# Autodesk Inventor assembly: Assembly1
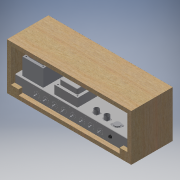
[picture p0: Inventor's stored thumbnail of the model, 180x180]
Saved by Autodesk Inventor 2016 (Build 200138000, 138)
## iProperties
Created: 2015-10-14
Part Number: Assembly1
Document SubType Name: Assembly
Designer: jeremyhale
Author: jeremyhale
## Documents named in this file (22)
- \\psf\Home\Documents\Poorhouse\git\p0001\Assembly1.iam
- \\psf\Home\Documents\Poorhouse\git\p0001\chassis.ipt
- \\psf\Home\Documents\Poorhouse\git\p0001\tube socket 8 pin.ipt
- \\psf\Home\Documents\Poorhouse\git\p0001\tube socket 9 pin.ipt
- \\psf\Home\Documents\Poorhouse\git\p0001\xmfr power.ipt
- \\psf\Home\Documents\Poorhouse\git\p0001\xmfr output.ipt
- \\psf\Home\Documents\Inventor\Content Center Files\R2016\en-US\AS 1427(08)\AS 1427 - M3 x 5(6) I.ipt
- \\psf\Home\Documents\Inventor\Content Center Files\R2016\en-US\AS 1474(1)\AS 1474 - M2.5(1).ipt
- \\psf\Home\Documents\Inventor\Content Center Files\R2016\en-US\AS 1474(1)\AS 1474 - M3.5(1).ipt
- \\psf\Home\Documents\Inventor\Content Center Files\R2016\en-US\AS 1474(1)\AS 1474 - M3(1).ipt
- \\psf\Home\Documents\Poorhouse\git\p0001\cabinet.ipt
- \\psf\Home\Documents\Poorhouse\git\p0001\iec320_703W-00_04.ipt
- \\psf\Home\Documents\Inventor\Content Center Files\R2016\en-US\AS 1427(07)\AS 1427 - M3 x 10(6) II.ipt
- \\psf\Home\Documents\Poorhouse\git\p0001\Toggle Large A.ipt
- \\psf\Home\Documents\Poorhouse\git\p0001\AUDIO JACK 2.ipt
- \\psf\Home\Documents\Poorhouse\git\p0001\12ax7_complete.ipt
- \\psf\Home\Documents\Poorhouse\git\p0001\Noval socket.ipt
- \\psf\Home\Documents\Poorhouse\git\p0001\octal assembly.ipt
- \\psf\Home\Documents\Poorhouse\git\p0001\el34 assembly_r1.ipt
- \\psf\Home\Documents\Poorhouse\git\p0001\rotary control.iam
- \\psf\Home\Documents\Poorhouse\git\p0001\Bussman fuse holder HKP - 0,25'' X 1,25''.ipt
- \\psf\Home\Documents\Poorhouse\git\p0001\cage nut m6.ipt
## Components (94 placed, 25 different names)
1. chassis:1 — Rotational:1, Rotational:2, Rotational:3, Rotational:4, Rotational:5, Rotational:6, Rotational:7, Rotational:8, Rotational:9, Rotational:10, Mate:4, Insert:20, Insert:21, Insert:22, Insert:23, Insert:24, Insert:25, Insert:26, Insert:27, Insert:28, Insert:29, Insert:30, Insert:31, Insert:32, Insert:33, Insert:34, Insert:35, Insert:36, Insert:37, Flush:1, Mate:5, Flush:2, Rotational:11, Rotational:12, Mate:11, Mate:13, Rigid:15, Rigid:18, Rigid:19, Rigid:20, Rotational:15, Rotational:16, Rotational:17, Rotational:18, Rotational:19, Rotational:20, Rotational:26, Rotational:27, Rigid:22, Rigid:23, Rigid:24, Rigid:25, Rigid:26
2. big preamp tube sockets — Rotational:3, Rotational:4, Insert:13, Insert:14
3. xmfr power:1 — Rotational:7, Rotational:8
4. xmfr output:1 — Rotational:9, Rotational:10
5. cabinet:1 — Flush:1, Mate:5, Flush:2
6. PowerSwitch — Rigid:23
7. Bussman fuse holder HKP - 0,25'' X 1,25'':1 — Rigid:22
8. Input Jack — Rotational:26
9. AS 1427 Z - Metric M3 x 5:1 — Insert:1, Mate:3
10. AS 1427 Z - Metric M3 x 5:2 — Insert:2
11. AS 1427 Z - Metric M3 x 5:3 — Insert:3
12. AS 1427 Z - Metric M3 x 5:4 — Insert:4
13. AS 1427 Z - Metric M3 x 5:5 — Insert:5
14. AS 1427 Z - Metric M3 x 5:6 — Insert:6
15. AS 1427 Z - Metric M3 x 5:7 — Insert:7
16. AS 1427 Z - Metric M3 x 5:8 — Insert:8
17. AS 1427 Z - Metric M3 x 5:9 — Insert:9
18. AS 1427 Z - Metric M3 x 5:10 — Insert:10
19. AS 1427 Z - Metric M3 x 5:11 — Insert:11
20. AS 1427 Z - Metric M3 x 5:12 — Insert:12
21. AS 1427 Z - Metric M3 x 5:13 — Insert:13
22. AS 1427 Z - Metric M3 x 5:14 — Insert:14
23. AS 1427 Z - Metric M3 x 5:15 — Insert:15
24. AS 1427 Z - Metric M3 x 5:16 — Insert:16
25. AS 1427 Z - Metric M3 x 5:17 — Insert:17
26. AS 1427 Z - Metric M3 x 5:18 — Insert:18
27. AS 1474 - Metric M2.5:1 — Mate:3, Mate:4
28. AS 1474 - Metric M3.5:1 — Insert:20
29. AS 1474 - Metric M3.5:2 — Insert:21
30. AS 1474 - Metric M3.5:3 — Insert:22
31. AS 1474 - Metric M3.5:4 — Insert:23
32. AS 1474 - Metric M3.5:5 — Insert:24
33. AS 1474 - Metric M3.5:6 — Insert:25
34. AS 1474 - Metric M3.5:7 — Insert:26
35. AS 1474 - Metric M3.5:8 — Insert:27
36. AS 1474 - Metric M3.5:9 — Insert:28
37. AS 1474 - Metric M3.5:10 — Insert:29
38. AS 1474 - Metric M3.5:11 — Insert:30
39. AS 1474 - Metric M3.5:12 — Insert:31
40. AS 1474 - Metric M3.5:13 — Insert:32
41. AS 1474 - Metric M3.5:14 — Insert:33
42. AS 1474 - Metric M3:1 — Insert:34
43. AS 1474 - Metric M3:2 — Insert:35
44. AS 1474 - Metric M3:3 — Insert:36
45. AS 1474 - Metric M3:4 — Insert:37
46. iec320_703W-00_04:1 — Rotational:11, Rotational:12, Mate:6, Mate:7
47. AS 1427 Z - Metric M3 x 10:2 — Mate:6, Mate:10
48. AS 1427 Z - Metric M3 x 10:1 — Mate:7, Mate:12
49. AS 1474 - Metric M3:5 — Mate:10, Mate:11
50. AS 1474 - Metric M3:6 — Mate:12, Mate:13
51. 12ax7_complete:1 — Rotational:13
52. 12ax7_complete:2 — Rotational:14
53. Noval socket:1 — Rigid:18, Rotational:13
54. Noval socket:2 — Rigid:19, Rotational:14
55. octal assembly:1 — Rigid:20
56. octal assembly:2 — Rotational:15, Rotational:21
57. octal assembly:3 — Rotational:16, Rotational:22
58. octal assembly:4 — Rotational:18, Rotational:23
59. octal assembly:5 — Rotational:17, Rigid:21
60. octal assembly:6 — Rotational:19, Rotational:24
61. octal assembly:7 — Rotational:20, Rotational:25
62. el34 assembly_r1:1 — Rotational:21
63. el34 assembly_r1:2 — Rotational:22
64. el34 assembly_r1:3 — Rigid:21
65. el34 assembly_r1:4 — Rotational:23
66. el34 assembly_r1:5 — Rotational:24
67. el34 assembly_r1:6 — Rotational:25
68. tube socket 8 pin:1 — Rotational:1, Rotational:2, Insert:1, Insert:2
69. tube socket 8 pin:2 — Insert:3, Insert:4
70. tube socket 8 pin:3 — Insert:5, Insert:6
71. tube socket 8 pin:4 — Insert:7, Insert:8
72. tube socket 8 pin:5 — Insert:15, Insert:16
73. tube socket 8 pin:6 — Insert:17, Insert:18
74. tube socket 9 pin:1 — Rotational:5, Rotational:6, Insert:9, Insert:10
75. tube socket 9 pin:2 — Insert:11, Insert:12
76. rotary control:1 [sub-assembly] — Rotational:27
77. rotary control:2 [sub-assembly]
78. rotary control:3 [sub-assembly]
79. rotary control:4 [sub-assembly]
80. rotary control:5 [sub-assembly]
81. rotary control:6 [sub-assembly]
82. rotary control:7 [sub-assembly]
83. rotary control:8 [sub-assembly]
84. Speaker — Rigid:15
85. AUDIO JACK 2:3
86. AUDIO JACK 2:4
87. cage nut cage — Rigid:24
88. cage nut m6:2
89. cage nut m6:3
90. cage nut m6:4
91. cage nut m6:5 — Rigid:25
92. cage nut m6:6
93. cage nut m6:7 — Rigid:26
94. cage nut m6:8
## Component patterns: Big Tube Sockets (6 elements), small preamp tube sockets (2 elements), Rotary Controls (8 elements), Speaker Jacks (3 elements), Cage Nuts Top (4 elements), Cage Nuts Side Right (2 elements), Cage Nuts Side Left (2 elements)
## Relationships (84: Insert 36, RevoluteJoint 27, WeldJoint 10, Mate 9, Flush 2)
- Rotational:1 [RevoluteJoint]: chassis:1 ↔ tube socket 8 pin:1
- Rotational:2 [RevoluteJoint]: chassis:1 ↔ tube socket 8 pin:1
- Rotational:3 [RevoluteJoint]: chassis:1 ↔ big preamp tube sockets
- Rotational:4 [RevoluteJoint]: chassis:1 ↔ big preamp tube sockets
- Rotational:5 [RevoluteJoint]: chassis:1 ↔ tube socket 9 pin:1
- Rotational:6 [RevoluteJoint]: chassis:1 ↔ tube socket 9 pin:1
- Rotational:7 [RevoluteJoint]: chassis:1 ↔ xmfr power:1
- Rotational:8 [RevoluteJoint]: chassis:1 ↔ xmfr power:1
- Rotational:9 [RevoluteJoint]: chassis:1 ↔ xmfr output:1
- Rotational:10 [RevoluteJoint]: chassis:1 ↔ xmfr output:1
- Insert:1: AS 1427 Z - Metric M3 x 5:1 ↔ tube socket 8 pin:1
- Insert:2: AS 1427 Z - Metric M3 x 5:2 ↔ tube socket 8 pin:1
- Insert:3: AS 1427 Z - Metric M3 x 5:3 ↔ tube socket 8 pin:2
- Insert:4: AS 1427 Z - Metric M3 x 5:4 ↔ tube socket 8 pin:2
- Insert:5: AS 1427 Z - Metric M3 x 5:5 ↔ tube socket 8 pin:3
- Insert:6: AS 1427 Z - Metric M3 x 5:6 ↔ tube socket 8 pin:3
- Insert:7: AS 1427 Z - Metric M3 x 5:7 ↔ tube socket 8 pin:4
- Insert:8: AS 1427 Z - Metric M3 x 5:8 ↔ tube socket 8 pin:4
- Insert:9: AS 1427 Z - Metric M3 x 5:9 ↔ tube socket 9 pin:1
- Insert:10: AS 1427 Z - Metric M3 x 5:10 ↔ tube socket 9 pin:1
- Insert:11: AS 1427 Z - Metric M3 x 5:11 ↔ tube socket 9 pin:2
- Insert:12: AS 1427 Z - Metric M3 x 5:12 ↔ tube socket 9 pin:2
- Insert:13: big preamp tube sockets ↔ AS 1427 Z - Metric M3 x 5:13
- Insert:14: big preamp tube sockets ↔ AS 1427 Z - Metric M3 x 5:14
- Insert:15: AS 1427 Z - Metric M3 x 5:15 ↔ tube socket 8 pin:5
- Insert:16: AS 1427 Z - Metric M3 x 5:16 ↔ tube socket 8 pin:5
- Insert:17: AS 1427 Z - Metric M3 x 5:17 ↔ tube socket 8 pin:6
- Insert:18: AS 1427 Z - Metric M3 x 5:18 ↔ tube socket 8 pin:6
- Mate:3: AS 1427 Z - Metric M3 x 5:1 ↔ AS 1474 - Metric M2.5:1
- Mate:4: chassis:1 ↔ AS 1474 - Metric M2.5:1
- Insert:20: chassis:1 ↔ AS 1474 - Metric M3.5:1
- Insert:21: chassis:1 ↔ AS 1474 - Metric M3.5:2
- Insert:22: chassis:1 ↔ AS 1474 - Metric M3.5:3
- Insert:23: chassis:1 ↔ AS 1474 - Metric M3.5:4
- Insert:24: chassis:1 ↔ AS 1474 - Metric M3.5:5
- Insert:25: chassis:1 ↔ AS 1474 - Metric M3.5:6
- Insert:26: chassis:1 ↔ AS 1474 - Metric M3.5:7
- Insert:27: chassis:1 ↔ AS 1474 - Metric M3.5:8
- Insert:28: chassis:1 ↔ AS 1474 - Metric M3.5:9
- Insert:29: chassis:1 ↔ AS 1474 - Metric M3.5:10
- Insert:30: chassis:1 ↔ AS 1474 - Metric M3.5:11
- Insert:31: chassis:1 ↔ AS 1474 - Metric M3.5:12
- Insert:32: chassis:1 ↔ AS 1474 - Metric M3.5:13
- Insert:33: chassis:1 ↔ AS 1474 - Metric M3.5:14
- Insert:34: chassis:1 ↔ AS 1474 - Metric M3:1
- Insert:35: chassis:1 ↔ AS 1474 - Metric M3:2
- Insert:36: chassis:1 ↔ AS 1474 - Metric M3:3
- Insert:37: chassis:1 ↔ AS 1474 - Metric M3:4
- Flush:1: chassis:1 ↔ cabinet:1
- Mate:5: chassis:1 ↔ cabinet:1
- Flush:2 (-19.05 mm): chassis:1 ↔ cabinet:1
- Rotational:11 [RevoluteJoint]: chassis:1 ↔ iec320_703W-00_04:1
- Rotational:12 [RevoluteJoint]: chassis:1 ↔ iec320_703W-00_04:1
- Mate:6: iec320_703W-00_04:1 ↔ AS 1427 Z - Metric M3 x 10:2
- Mate:7: iec320_703W-00_04:1 ↔ AS 1427 Z - Metric M3 x 10:1
- Mate:10: AS 1427 Z - Metric M3 x 10:2 ↔ AS 1474 - Metric M3:5
- Mate:11: chassis:1 ↔ AS 1474 - Metric M3:5
- Mate:12: AS 1427 Z - Metric M3 x 10:1 ↔ AS 1474 - Metric M3:6
- Mate:13: chassis:1 ↔ AS 1474 - Metric M3:6
- Rigid:15 [WeldJoint]: chassis:1 ↔ Speaker
- Rigid:18 [WeldJoint]: chassis:1 ↔ Noval socket:1
- Rigid:19 [WeldJoint]: chassis:1 ↔ Noval socket:2
- Rotational:13 [RevoluteJoint]: 12ax7_complete:1 ↔ Noval socket:1
- Rotational:14 [RevoluteJoint]: 12ax7_complete:2 ↔ Noval socket:2
- Rigid:20 [WeldJoint]: chassis:1 ↔ octal assembly:1
- Rotational:15 [RevoluteJoint]: chassis:1 ↔ octal assembly:2
- Rotational:16 [RevoluteJoint]: chassis:1 ↔ octal assembly:3
- Rotational:17 [RevoluteJoint]: chassis:1 ↔ octal assembly:5
- Rotational:18 [RevoluteJoint]: chassis:1 ↔ octal assembly:4
- Rotational:19 [RevoluteJoint]: chassis:1 ↔ octal assembly:6
- Rotational:20 [RevoluteJoint]: chassis:1 ↔ octal assembly:7
- Rotational:21 [RevoluteJoint]: octal assembly:2 ↔ el34 assembly_r1:1
- Rotational:22 [RevoluteJoint]: octal assembly:3 ↔ el34 assembly_r1:2
- Rigid:21 [WeldJoint]: octal assembly:5 ↔ el34 assembly_r1:3
- Rotational:23 [RevoluteJoint]: octal assembly:4 ↔ el34 assembly_r1:4
- Rotational:24 [RevoluteJoint]: octal assembly:6 ↔ el34 assembly_r1:5
- Rotational:25 [RevoluteJoint]: octal assembly:7 ↔ el34 assembly_r1:6
- Rotational:26 [RevoluteJoint]: chassis:1 ↔ Input Jack
- Rotational:27 [RevoluteJoint]: chassis:1 ↔ rotary control:1
- Rigid:22 [WeldJoint]: chassis:1 ↔ Bussman fuse holder HKP - 0,25'' X 1,25'':1
- Rigid:23 [WeldJoint]: chassis:1 ↔ PowerSwitch
- Rigid:24 [WeldJoint]: chassis:1 ↔ cage nut cage
- Rigid:25 [WeldJoint]: chassis:1 ↔ cage nut m6:5
- Rigid:26 [WeldJoint]: chassis:1 ↔ cage nut m6:7
## Named parameters: ControlSpacing = 44.45 mm
